# Autodesk Inventor assembly: Frame
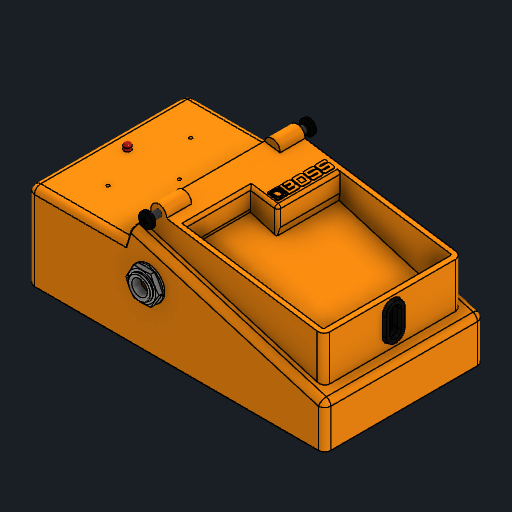
[picture p0: Inventor's stored thumbnail of the model, 512x512]
Saved by Autodesk Inventor 2026.2 (Build 302298000, 298)
## iProperties
Created: 2026-06-03
Part Number: Frame
Document SubType Name: Assembly
Designer: JoshuaEah
Author: JoshuaEah
## Documents named in this file (9)
- C:\Users\JoshuaEah\Documents\GitHub\Designed-Trinkets\Guitar\Modular Pedalboard\Pedals\Boss Pedal\Frame.iam
- C:\Users\JoshuaEah\Documents\GitHub\Designed-Trinkets\Guitar\Modular Pedalboard\Pedals\Boss Pedal\Frame.ipt
- C:\Users\JoshuaEah\Documents\GitHub\Designed-Trinkets\Guitar\Modular Pedalboard\Pedals\Boss Pedal\Washer.ipt
- C:\Users\JoshuaEah\Documents\GitHub\Designed-Trinkets\Guitar\Modular Pedalboard\Pedals\Boss Pedal\Rod.ipt
- C:\Users\JoshuaEah\Documents\GitHub\Designed-Trinkets\Guitar\Modular Pedalboard\Pedals\Boss Pedal\Nut.ipt
- C:\Users\JoshuaEah\Documents\GitHub\Designed-Trinkets\Guitar\Modular Pedalboard\Pedals\Boss Pedal\Nibblets.ipt
- C:\Users\JoshuaEah\Documents\GitHub\Designed-Trinkets\Guitar\Modular Pedalboard\Pedals\Boss Pedal\Plug.ipt
- C:\Users\JoshuaEah\Documents\GitHub\Designed-Trinkets\Guitar\Modular Pedalboard\Pedals\Boss Pedal\Bottom.ipt
- C:\Users\JoshuaEah\Documents\GitHub\Designed-Trinkets\Guitar\Modular Pedalboard\Pedals\Boss Pedal\ANSI B18.6.3 - 4-48 UNF - 0.375(14).ipt
## Components (16 placed, 8 different names)
1. Frame:1 — Insert:7, Insert:9, Insert:10, Rigid:1, Mate:1, Slider:1
2. Washer:1 — Insert:7
3. Washer:2 — Insert:8, Insert:9
4. Rod:1
5. Rod:2 — Insert:8
6. Nut:1
7. Nut:2
8. Nibblets:1 — Insert:10
9. Plug:1 — Rigid:1
10. Bottom:1 — Mate:1, Slider:1
11. ANSI B18.6.3 - 4-48 UNF - 0.375(14):3
12. ANSI B18.6.3 - 4-48 UNF - 0.375(14):4
13. ANSI B18.6.3 - 4-48 UNF - 0.375(14):5
14. ANSI B18.6.3 - 4-48 UNF - 0.375(14):6
15. ANSI B18.6.3 - 4-48 UNF - 0.375(14):1
16. ANSI B18.6.3 - 4-48 UNF - 0.375(14):2
## Relationships (12: Insert 9, WeldJoint 1, Mate 1, TranslationJoint 1)
- [Insert]: Washer:1 ↔ Rod:1
- [Insert]: Washer:1 ↔ Nut:1
- [Insert]: Washer:2 ↔ Nut:2
- Insert:7: Frame:1 ↔ Washer:1
- Insert:8: Washer:2 ↔ Rod:2
- Insert:9: Frame:1 ↔ Washer:2
- Insert:10: Frame:1 ↔ Nibblets:1
- Rigid:1 [WeldJoint]: Frame:1 ↔ Plug:1
- Mate:1: Frame:1 ↔ Bottom:1
- Slider:1 [TranslationJoint]: Frame:1 ↔ Bottom:1
- [Insert]: Frame:1 ↔ ANSI B18.6.3 - 4-48 UNF - 0.375(14):5
- [Insert]: Frame:1 ↔ ANSI B18.6.3 - 4-48 UNF - 0.375(14):4
## Named parameters: d0_d4 = 0 mm, d1_d5 = 0 mm
